# Autodesk Inventor assembly: 160203GearSet
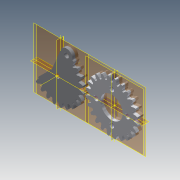
[picture p0: Inventor's stored thumbnail of the model, 180x180]
Saved by Autodesk Inventor 2015 SP1 (Build 190203100, 203)
## iProperties
Created: 2015-11-20
Part Number: 160203GearSet
Document SubType Name: Assembly
Designer: Yamaura
Author: Yamaura
## Documents named in this file (3)
- C:\Users\Yamaura\Documents\GitHub\HACKberry\HACKberry-hardware\3D\Inventor\Parts\160203GearSet.iam
- C:\Users\Yamaura\Documents\GitHub\HACKberry\HACKberry-hardware\3D\Inventor\Parts\HbIndexInputLink02.ipt
- C:\Users\Yamaura\Documents\GitHub\HACKberry\HACKberry-hardware\3D\Inventor\Parts\HbIndexMotorGear02.ipt
## Components (2 placed, 2 different names)
1. HbIndexMotorGear02:1 — フラッシュ:4, メイト:1, メイト:2
2. HbIndexInputLink02:1 — フラッシュ:1, フラッシュ:2, フラッシュ:3, フラッシュ:4
## Relationships (6: Flush 4, Mate 2)
- フラッシュ:1 [Flush]: HbIndexInputLink02:1
- フラッシュ:2 [Flush]: HbIndexInputLink02:1
- フラッシュ:3 [Flush]: HbIndexInputLink02:1
- フラッシュ:4 [Flush]: HbIndexMotorGear02:1 ↔ HbIndexInputLink02:1
- メイト:1 [Mate]: HbIndexMotorGear02:1
- メイト:2 [Mate] (27 mm): HbIndexMotorGear02:1
